# Autodesk Inventor assembly: Banda completa
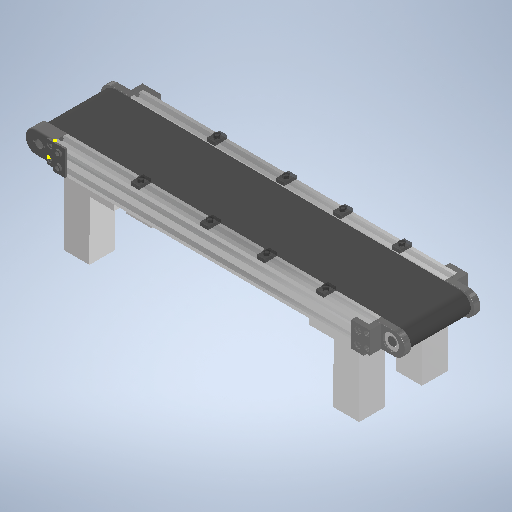
[picture p0: Inventor's stored thumbnail of the model, 512x512]
Saved by Autodesk Inventor 2025 (Build 290162000, 162)
## iProperties
Created: 2026-09-21
Part Number: Banda completa
Document SubType Name: Assembly
Designer: ASUS
Author: ASUS
## Documents named in this file (14)
- C:\Users\ASUS\Desktop\Partes Banda Transportadora\Banda completa.iam
- C:\Users\ASUS\Desktop\Partes Banda Transportadora\Riel Banda.ipt
- C:\Users\ASUS\Desktop\Partes Banda Transportadora\Pata1.ipt
- C:\Users\ASUS\Desktop\Partes Banda Transportadora\Pata2.ipt
- C:\Users\ASUS\Desktop\Partes Banda Transportadora\palito arriba de la banda.ipt
- C:\Users\ASUS\Desktop\Partes Banda Transportadora\Pieza negra.ipt
- C:\Users\ASUS\Desktop\Partes Banda Transportadora\pieza negra derecha.ipt
- C:\Users\ASUS\Desktop\Partes Banda Transportadora\BaseRodamiento.ipt
- C:\Users\ASUS\Desktop\Partes Banda Transportadora\Base Rodamiento delgado.ipt
- C:\Users\ASUS\Desktop\Partes Banda Transportadora\Rodamiento grande.ipt
- C:\Users\ASUS\Desktop\Partes Banda Transportadora\rodillo con rodamiento.ipt
- C:\Users\ASUS\Desktop\Partes Banda Transportadora\rodamiento.ipt
- C:\Users\ASUS\Desktop\Partes Banda Transportadora\rodillo con rodamiento 2.ipt
- C:\Users\ASUS\Desktop\Partes Banda Transportadora\Banda.ipt
## Components (25 placed, 13 different names)
1. Riel Banda:1 — Nivelación:5, Nivelación:6, Coincidencia:3, Coincidencia:5, Nivelación:9, Nivelación:10, Coincidencia:6, Nivelación:13, Nivelación:14, Nivelación:16, Nivelación:17, Coincidencia:8, Nivelación:20, Nivelación:21, Coincidencia:12, Nivelación:23, Coincidencia:13, Coincidencia:14, Nivelación:24, Coincidencia:15, Coincidencia:19, Coincidencia:20, Coincidencia:29, Nivelación:32
2. Riel Banda:2 — Coincidencia:2, Nivelación:3, Nivelación:4, Coincidencia:4, Nivelación:7, Nivelación:8, Nivelación:12, Nivelación:13, Nivelación:15, Coincidencia:7, Nivelación:18, Nivelación:19, Coincidencia:9, Coincidencia:10, Nivelación:22, Coincidencia:11, Coincidencia:22, Coincidencia:25, Nivelación:29, Coincidencia:26, Nivelación:30, Nivelación:31, Coincidencia:27
3. Pata1:1 — Coincidencia:5, Nivelación:9, Nivelación:10
4. Pata1:2 — Coincidencia:2, Nivelación:3, Nivelación:4, Nivelación:11
5. Pata2:1 — Coincidencia:4, Nivelación:7, Nivelación:8
6. Pata2:2 — Nivelación:5, Nivelación:6, Coincidencia:3, Nivelación:11
7. palito arriba de la banda:1 — Coincidencia:6, Nivelación:12, Nivelación:14, Nivelación:15
8. palito arriba de la banda:2 — Coincidencia:8, Nivelación:18, Nivelación:19
9. palito arriba de la banda:3 — Coincidencia:7, Nivelación:16, Nivelación:17
10. palito arriba de la banda:4 — Coincidencia:9, Nivelación:20, Nivelación:21
11. Pieza negra:1 — Coincidencia:10, Nivelación:22, Coincidencia:11, Coincidencia:21, Nivelación:27
12. Pieza negra:2 — Coincidencia:12, Nivelación:23, Coincidencia:13, Coincidencia:30
13. pieza negra derecha:2 — Coincidencia:14, Nivelación:24, Coincidencia:15, Coincidencia:18, Nivelación:26
14. BaseRodamiento:1 — Coincidencia:18, Coincidencia:19, Nivelación:26, Coincidencia:20
15. BaseRodamiento:5 — Coincidencia:21, Nivelación:27, Coincidencia:22, Coincidencia:33, Coincidencia:34
16. Base Rodamiento delgado:1 — Coincidencia:25, Nivelación:29, Nivelación:30, Coincidencia:28
17. Rodamiento grande:1 — Coincidencia:26, Nivelación:31, Coincidencia:27, Coincidencia:28
18. rodillo con rodamiento:1 — De rotación:1, De rotación:2, Coincidencia:35
19. rodamiento:1 — De rotación:1
20. rodamiento:2 — De rotación:2, Coincidencia:31, Coincidencia:32
21. BaseRodamiento:6 — Coincidencia:29, Nivelación:32, Coincidencia:30, Coincidencia:31, Coincidencia:32
22. rodillo con rodamiento 2:1 — De rotación:3, De rotación:4, Coincidencia:36, Coincidencia:37
23. rodamiento:3 — De rotación:3, Coincidencia:33, Coincidencia:34
24. rodamiento:4 — De rotación:4
25. Banda:1 — Coincidencia:35, Coincidencia:36, Coincidencia:37
## Relationships (64: Mate 32, Flush 28, RevoluteJoint 4)
- Coincidencia:2 [Mate]: Riel Banda:2 ↔ Pata1:2
- Nivelación:3 [Flush]: Riel Banda:2 ↔ Pata1:2
- Nivelación:4 [Flush] (-15 mm): Riel Banda:2 ↔ Pata1:2
- Nivelación:5 [Flush] (15 mm): Riel Banda:1 ↔ Pata2:2
- Nivelación:6 [Flush]: Riel Banda:1 ↔ Pata2:2
- Coincidencia:3 [Mate]: Riel Banda:1 ↔ Pata2:2
- Coincidencia:4 [Mate]: Riel Banda:2 ↔ Pata2:1
- Nivelación:7 [Flush]: Riel Banda:2 ↔ Pata2:1
- Nivelación:8 [Flush] (-15 mm): Riel Banda:2 ↔ Pata2:1
- Coincidencia:5 [Mate]: Riel Banda:1 ↔ Pata1:1
- Nivelación:9 [Flush]: Riel Banda:1 ↔ Pata1:1
- Nivelación:10 [Flush] (-15 mm): Riel Banda:1 ↔ Pata1:1
- Nivelación:11 [Flush]: Pata1:2 ↔ Pata2:2
- Coincidencia:6 [Mate]: Riel Banda:1 ↔ palito arriba de la banda:1
- Nivelación:12 [Flush]: Riel Banda:2 ↔ palito arriba de la banda:1
- Nivelación:13 [Flush]: Riel Banda:1 ↔ Riel Banda:2
- Nivelación:14 [Flush]: Riel Banda:1 ↔ palito arriba de la banda:1
- Nivelación:15 [Flush] (72 mm): Riel Banda:2 ↔ palito arriba de la banda:1
- Coincidencia:7 [Mate]: Riel Banda:2 ↔ palito arriba de la banda:3
- Nivelación:16 [Flush]: Riel Banda:1 ↔ palito arriba de la banda:3
- Nivelación:17 [Flush] (166 mm): Riel Banda:1 ↔ palito arriba de la banda:3
- Coincidencia:8 [Mate]: Riel Banda:1 ↔ palito arriba de la banda:2
- Nivelación:18 [Flush]: Riel Banda:2 ↔ palito arriba de la banda:2
- Nivelación:19 [Flush] (256 mm): Riel Banda:2 ↔ palito arriba de la banda:2
- Coincidencia:9 [Mate]: Riel Banda:2 ↔ palito arriba de la banda:4
- Nivelación:20 [Flush]: Riel Banda:1 ↔ palito arriba de la banda:4
- Nivelación:21 [Flush] (366 mm): Riel Banda:1 ↔ palito arriba de la banda:4
- Coincidencia:10 [Mate]: Riel Banda:2 ↔ Pieza negra:1
- Nivelación:22 [Flush]: Riel Banda:2 ↔ Pieza negra:1
- Coincidencia:11 [Mate]: Riel Banda:2 ↔ Pieza negra:1
- Coincidencia:12 [Mate]: Riel Banda:1 ↔ Pieza negra:2
- Nivelación:23 [Flush]: Riel Banda:1 ↔ Pieza negra:2
- Coincidencia:13 [Mate]: Riel Banda:1 ↔ Pieza negra:2
- Coincidencia:14 [Mate]: Riel Banda:1 ↔ pieza negra derecha:2
- Nivelación:24 [Flush]: Riel Banda:1 ↔ pieza negra derecha:2
- Coincidencia:15 [Mate]: Riel Banda:1 ↔ pieza negra derecha:2
- Coincidencia:18 [Mate]: pieza negra derecha:2 ↔ BaseRodamiento:1
- Coincidencia:19 [Mate]: Riel Banda:1 ↔ BaseRodamiento:1
- Nivelación:26 [Flush]: pieza negra derecha:2 ↔ BaseRodamiento:1
- Coincidencia:20 [Mate]: Riel Banda:1 ↔ BaseRodamiento:1
- Coincidencia:21 [Mate]: Pieza negra:1 ↔ BaseRodamiento:5
- Nivelación:27 [Flush]: Pieza negra:1 ↔ BaseRodamiento:5
- Coincidencia:22 [Mate]: Riel Banda:2 ↔ BaseRodamiento:5
- Coincidencia:25 [Mate]: Riel Banda:2 ↔ Base Rodamiento delgado:1
- Nivelación:29 [Flush]: Riel Banda:2 ↔ Base Rodamiento delgado:1
- Coincidencia:26 [Mate]: Riel Banda:2 ↔ Rodamiento grande:1
- Nivelación:30 [Flush]: Riel Banda:2 ↔ Base Rodamiento delgado:1
- Nivelación:31 [Flush]: Riel Banda:2 ↔ Rodamiento grande:1
- Coincidencia:27 [Mate]: Riel Banda:2 ↔ Rodamiento grande:1
- Coincidencia:28 [Mate]: Base Rodamiento delgado:1 ↔ Rodamiento grande:1
- De rotación:1 [RevoluteJoint]: rodillo con rodamiento:1 ↔ rodamiento:1
- De rotación:2 [RevoluteJoint]: rodillo con rodamiento:1 ↔ rodamiento:2
- Coincidencia:29 [Mate]: Riel Banda:1 ↔ BaseRodamiento:6
- Nivelación:32 [Flush]: Riel Banda:1 ↔ BaseRodamiento:6
- Coincidencia:30 [Mate]: Pieza negra:2 ↔ BaseRodamiento:6
- Coincidencia:31 [Mate]: rodamiento:2 ↔ BaseRodamiento:6
- Coincidencia:32 [Mate]: rodamiento:2 ↔ BaseRodamiento:6
- De rotación:3 [RevoluteJoint]: rodillo con rodamiento 2:1 ↔ rodamiento:3
- De rotación:4 [RevoluteJoint]: rodillo con rodamiento 2:1 ↔ rodamiento:4
- Coincidencia:33 [Mate]: BaseRodamiento:5 ↔ rodamiento:3
- Coincidencia:34 [Mate]: BaseRodamiento:5 ↔ rodamiento:3
- Coincidencia:35 [Mate]: rodillo con rodamiento:1 ↔ Banda:1
- Coincidencia:36 [Mate]: rodillo con rodamiento 2:1 ↔ Banda:1
- Coincidencia:37 [Mate]: rodillo con rodamiento 2:1 ↔ Banda:1
